# Autodesk Inventor assembly: Assy_arm_connection
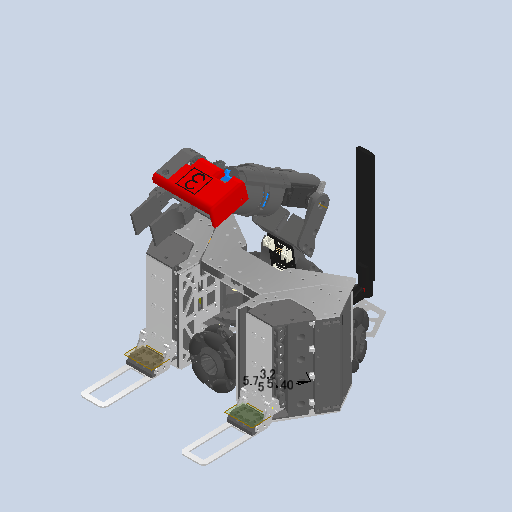
[picture p0: Inventor's stored thumbnail of the model, 512x512]
Saved by Autodesk Inventor 2024.1 (Build 281209000, 209)
## iProperties
Created: 2025-03-04
Part Number: Assy_arm_connection
Document SubType Name: Assembly
Designer: hibik
Author: hibik
## Documents named in this file (3)
- C:\Users\hibik\Documents\Robomech\RESCUE\ORCA\hard\Assy_arm_connection.iam
- C:\Users\hibik\Documents\Robomech\RESCUE\ORCA\hard\Assy_fork_connection.iam
- C:\Users\hibik\Documents\Robomech\RESCUE\ORCA\hard\arm\Assy_arm.iam
## Components (2 placed, 2 different names)
1. Assy_fork_connection:1 [sub-assembly] — 挿入:17, 挿入:18
2. Assy_arm:1 [sub-assembly] — 挿入:17, 挿入:18
## Relationships (2: Insert 2)
- 挿入:17 [Insert]: Assy_fork_connection:1 ↔ Assy_arm:1
- 挿入:18 [Insert]: Assy_fork_connection:1 ↔ Assy_arm:1
